# Autodesk Inventor assembly: 001_Khung_nhom
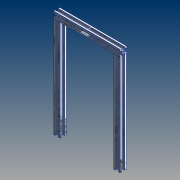
[picture p0: Inventor's stored thumbnail of the model, 180x180]
Saved by Autodesk Inventor 2021 (Build 250183000, 183)
## iProperties
Created: 2024-04-04
Part Number: 001_Khung_nhom
Document SubType Name: Assembly
Designer: Admin
Author: Admin
## Documents named in this file (3)
- C:\Users\Admin\Desktop\DO_AN_TOT_NGHIEP_2024\Mechanical\Design_in_3D\Version_1\001_Khung_nhom.iam
- C:\Users\Admin\Desktop\DO_AN_TOT_NGHIEP_2024\Mechanical\Design_in_3D\Library\khung-nhom-d-nh-hinh-trong-cong-nghi-p-1.snapshot.1\Modify_Ky_Anh\20x20x200.ipt
- C:\Users\Admin\Desktop\DO_AN_TOT_NGHIEP_2024\Mechanical\Design_in_3D\Library\khung-nhom-d-nh-hinh-trong-cong-nghi-p-1.snapshot.1\Modify_Ky_Anh\20x20x300.ipt
## Components (3 placed, 2 different names)
1. 20x20x200:1 — Mate:1, Flush:1, Mate:2, Flush:2, Flush:3, Flush:4
2. 20x20x300:1 — Mate:1, Flush:3, Flush:4
3. 20x20x300:2 — Flush:1, Mate:2, Flush:2
## Relationships (6: Flush 4, Mate 2)
- Mate:1: 20x20x200:1 ↔ 20x20x300:1
- Flush:1: 20x20x200:1 ↔ 20x20x300:2
- Mate:2: 20x20x200:1 ↔ 20x20x300:2
- Flush:2: 20x20x200:1 ↔ 20x20x300:2
- Flush:3: 20x20x200:1 ↔ 20x20x300:1
- Flush:4: 20x20x200:1 ↔ 20x20x300:1
